# Autodesk Inventor assembly: Robot Triciclo - Ensamble
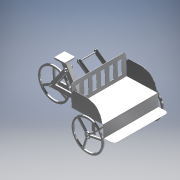
[picture p0: Inventor's stored thumbnail of the model, 180x180]
Saved by Autodesk Inventor 2019 (Build 230136000, 136)
## iProperties
Created: 2019-11-14
Part Number: Robot Triciclo - Ensamble
Document SubType Name: Weldment
Designer: eddysanoli
Weld Material: Welded Aluminum-6061
Author: eddysanoli
## Documents named in this file (13)
- E:\Archivos\Diseño\Inventor\Diseño Mecánico II\Proyecto - Triciclo\Mecanismos_Diseno\Robot Triciclo - Ensamble.iam
- E:\Archivos\Diseño\Inventor\Diseño Mecánico II\Proyecto - Triciclo\Mecanismos_Diseno\Asiento - Ensamble.iam
- E:\Archivos\Diseño\Inventor\Diseño Mecánico II\Proyecto - Triciclo\Mecanismos_Diseno\Marco_triciclo.iam
- E:\Archivos\Diseño\Inventor\Diseño Mecánico II\Proyecto - Triciclo\Mecanismos_Diseno\Rueda_triciclo.ipt
- E:\Archivos\Diseño\Inventor\Diseño Mecánico II\Proyecto - Triciclo\Mecanismos_Diseno\Pedal.ipt
- E:\Archivos\Diseño\Inventor\Diseño Mecánico II\Proyecto - Triciclo\Mecanismos_Diseno\Robot Triciclo - Ensamble\Design Accelerator\Eje1.iam
- E:\Archivos\Diseño\Inventor\Diseño Mecánico II\Proyecto - Triciclo\Mecanismos_Diseno\Marco - Asiento Triciclo.ipt
- E:\Archivos\Diseño\Inventor\Diseño Mecánico II\Proyecto - Triciclo\Mecanismos_Diseno\Robot Triciclo - Ensamble\Design Accelerator\Chain Drive1.iam
- E:\Archivos\Diseño\Inventor\Diseño Mecánico II\Proyecto - Triciclo\Mecanismos_Diseno\librarie\en-US\ANSI B27.8M\ANSI B27.8M - 3DM1-3DM1-16.ipt
- E:\Archivos\Diseño\Inventor\Diseño Mecánico II\Proyecto - Triciclo\Mecanismos_Diseno\Robot Triciclo - Ensamble\Design Accelerator\Eje Pedales - Ensamblaje.iam
- E:\Archivos\Diseño\Inventor\Diseño Mecánico II\Proyecto - Triciclo\Mecanismos_Diseno\Robot Triciclo - Ensamble\Design Accelerator\Eje Pedales - Ensamblaje1.iam
- E:\Archivos\Diseño\Inventor\Diseño Mecánico II\Proyecto - Triciclo\Mecanismos_Diseno\librarie\en-US\ANSI B27.8M\ANSI B27.8M - 3DM1-3DM1-13.ipt
- E:\Archivos\Diseño\Inventor\Diseño Mecánico II\Proyecto - Triciclo\Mecanismos_Diseno\librarie\en-US\JIS B 1521\JIS B 1521 - 6802 15x24x5x2.07.ipt
## Components (16 placed, 12 different names)
1. Asiento - Ensamble:1 [sub-assembly] — Coincidencia:1, Coincidencia:2, Nivelación:1, Coincidencia:3, Coincidencia:4, Coincidencia:5, Coincidencia:6, Coincidencia:10
2. Marco_triciclo:2 [sub-assembly] — Coincidencia:1, Coincidencia:2, Nivelación:1, Coincidencia:7, Coincidencia:8, Coincidencia:9, Coincidencia:11, Nivelación:4, Nivelación:5, Mate:16, Flush:8, Mate:18, Mate:26
3. Rueda_triciclo:1 — Coincidencia:3, Coincidencia:5
4. Rueda_triciclo:2 — Coincidencia:4, Coincidencia:6, Nivelación:3
5. Pedal:1 — Nivelación:2, Coincidencia:7, Coincidencia:9, Flush:6
6. Pedal:2 — Nivelación:2, Coincidencia:8, Flush:7
7. Eje:1 [sub-assembly] — Coincidencia:10, Nivelación:3, Mate:12, Mate:13, Mate:14, Mate:15
8. Marco - Asiento Triciclo:1 — Coincidencia:11, Nivelación:4, Nivelación:5
9. Chain Drive:1 [sub-assembly] — Mate:17
10. ANSI B27.8M 3DM1-3DM1-16:1 — Mate:12, Mate:13
11. ANSI B27.8M 3DM1-3DM1-16:2 — Mate:14, Mate:15
12. Eje Pedales - Ensamblaje:1 [sub-assembly] — Mate:16, Flush:6, Flush:7, Mate:17
13. Eje Rueda Trasera - Ensamblaje:1 [sub-assembly] — Flush:8, Mate:18, Mate:21, Mate:22, Mate:23, Mate:24, Mate:25
14. ANSI B27.8M 3DM1-3DM1-13:1 — Mate:21, Mate:22
15. ANSI B27.8M 3DM1-3DM1-13:2 — Mate:23, Mate:24
16. JIS B 1521 6802 15x24x5:1 — Mate:25, Mate:26
## Relationships (32: Mate 24, Flush 8)
- Coincidencia:1 [Mate]: Asiento - Ensamble:1 ↔ Marco_triciclo:2
- Coincidencia:2 [Mate] (59.8 mm): Asiento - Ensamble:1 ↔ Marco_triciclo:2
- Nivelación:1 [Flush] (183.5 mm): Asiento - Ensamble:1 ↔ Marco_triciclo:2
- Coincidencia:3 [Mate]: Asiento - Ensamble:1 ↔ Rueda_triciclo:1
- Coincidencia:4 [Mate]: Asiento - Ensamble:1 ↔ Rueda_triciclo:2
- Coincidencia:5 [Mate] (35 mm): Asiento - Ensamble:1 ↔ Rueda_triciclo:1
- Coincidencia:6 [Mate] (35 mm): Asiento - Ensamble:1 ↔ Rueda_triciclo:2
- Nivelación:2 [Flush]: Pedal:1 ↔ Pedal:2
- Coincidencia:7 [Mate]: Marco_triciclo:2 ↔ Pedal:1
- Coincidencia:8 [Mate]: Marco_triciclo:2 ↔ Pedal:2
- Coincidencia:9 [Mate]: Marco_triciclo:2 ↔ Pedal:1
- Coincidencia:10 [Mate]: Asiento - Ensamble:1 ↔ Eje:1
- Nivelación:3 [Flush] (-2.5 mm): Rueda_triciclo:2 ↔ Eje:1
- Coincidencia:11 [Mate]: Marco_triciclo:2 ↔ Marco - Asiento Triciclo:1
- Nivelación:4 [Flush] (24 mm): Marco_triciclo:2 ↔ Marco - Asiento Triciclo:1
- Nivelación:5 [Flush] (-20 mm): Marco_triciclo:2 ↔ Marco - Asiento Triciclo:1
- Mate:12: Eje:1 ↔ ANSI B27.8M 3DM1-3DM1-16:1
- Mate:13: Eje:1 ↔ ANSI B27.8M 3DM1-3DM1-16:1
- Mate:14: Eje:1 ↔ ANSI B27.8M 3DM1-3DM1-16:2
- Mate:15: Eje:1 ↔ ANSI B27.8M 3DM1-3DM1-16:2
- Mate:16: Marco_triciclo:2 ↔ Eje Pedales - Ensamblaje:1
- Flush:6: Pedal:1 ↔ Eje Pedales - Ensamblaje:1
- Flush:7: Pedal:2 ↔ Eje Pedales - Ensamblaje:1
- Mate:17 (4.7 mm): Chain Drive:1 ↔ Eje Pedales - Ensamblaje:1
- Flush:8 (-1 mm): Marco_triciclo:2 ↔ Eje Rueda Trasera - Ensamblaje:1
- Mate:18: Marco_triciclo:2 ↔ Eje Rueda Trasera - Ensamblaje:1
- Mate:21: Eje Rueda Trasera - Ensamblaje:1 ↔ ANSI B27.8M 3DM1-3DM1-13:1
- Mate:22: Eje Rueda Trasera - Ensamblaje:1 ↔ ANSI B27.8M 3DM1-3DM1-13:1
- Mate:23: Eje Rueda Trasera - Ensamblaje:1 ↔ ANSI B27.8M 3DM1-3DM1-13:2
- Mate:24: Eje Rueda Trasera - Ensamblaje:1 ↔ ANSI B27.8M 3DM1-3DM1-13:2
- Mate:25: Eje Rueda Trasera - Ensamblaje:1 ↔ JIS B 1521 6802 15x24x5:1
- Mate:26: Marco_triciclo:2 ↔ JIS B 1521 6802 15x24x5:1
